# Autodesk Inventor assembly: Adrian_Box
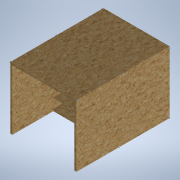
[picture p0: Inventor's stored thumbnail of the model, 180x180]
Saved by Autodesk Inventor 2021 (Build 250183000, 183)
## iProperties
Created: 2022-07-12
Part Number: Adrian_Box
Document SubType Name: Assembly
Designer: adria
Mass: 12178.9 g
Surface Area: 30264.5 cm^2
Volume: 21790.4 cm^3
Density: 0.55891 g/cm^3
Author: adria
## Documents named in this file (7)
- C:\Users\adria\OneDrive - tum.de\G2_Waste-Recycling\CAD\Adrian_Box.iam
- C:\Users\adria\OneDrive - tum.de\G2_Waste-Recycling\CAD\Seite_links.ipt
- C:\Users\adria\OneDrive - tum.de\G2_Waste-Recycling\CAD\Oben.ipt
- C:\Users\adria\OneDrive - tum.de\G2_Waste-Recycling\CAD\Seite.ipt
- C:\Users\adria\OneDrive - tum.de\G2_Waste-Recycling\CAD\Boden_drehscheibe.ipt
- C:\Users\adria\OneDrive - tum.de\G2_Waste-Recycling\CAD\Boden.ipt
- C:\Users\adria\Documents\Inventor\Content Center Files\R2021\de-DE\ANSI B18.3.1M(6)\ANSI B18.3.1M - M8x1,25 x 35(1).ipt
## Components (15 placed, 6 different names)
1. Seite_links:2 — Passend:1, Fluchtend:1, Fluchtend:2
2. Oben:1 — Passend:1, Fluchtend:1, Fluchtend:2, Fluchtend:3, Fluchtend:4, Passend:2
3. Seite:1 — Fluchtend:3, Fluchtend:4, Passend:2, Fluchtend:5, Passend:3, Fluchtend:6, Passend:4, Fluchtend:7, Passend:5, Passend:6, Passend:7, Passend:8, Passend:9, Passend:10, Passend:11, Passend:12, Passend:13, Passend:14, Fluchtend:8
4. Boden_drehscheibe:1 — Passend:4, Fluchtend:7, Passend:15
5. Boden:1 — Fluchtend:5, Passend:3, Fluchtend:6, Passend:15
6. Zylinderschraube mit geschmiedetem Innensechskant - Metrisch M8x1,25 x 35:6 — Passend:5, Passend:10
7. Zylinderschraube mit geschmiedetem Innensechskant - Metrisch M8x1,25 x 35:7 — Passend:6, Passend:11
8. Zylinderschraube mit geschmiedetem Innensechskant - Metrisch M8x1,25 x 35:8 — Passend:7, Passend:12
9. Zylinderschraube mit geschmiedetem Innensechskant - Metrisch M8x1,25 x 35:9 — Passend:9, Passend:14
10. Zylinderschraube mit geschmiedetem Innensechskant - Metrisch M8x1,25 x 35:10 — Passend:8, Passend:13
11. Zylinderschraube mit geschmiedetem Innensechskant - Metrisch M8x1,25 x 35:11
12. Zylinderschraube mit geschmiedetem Innensechskant - Metrisch M8x1,25 x 35:12
13. Zylinderschraube mit geschmiedetem Innensechskant - Metrisch M8x1,25 x 35:13
14. Zylinderschraube mit geschmiedetem Innensechskant - Metrisch M8x1,25 x 35:14
15. Zylinderschraube mit geschmiedetem Innensechskant - Metrisch M8x1,25 x 35:15
## Relationships (23: Mate 15, Flush 8)
- Passend:1 [Mate]: Seite_links:2 ↔ Oben:1
- Fluchtend:1 [Flush]: Seite_links:2 ↔ Oben:1
- Fluchtend:2 [Flush]: Seite_links:2 ↔ Oben:1
- Fluchtend:3 [Flush]: Oben:1 ↔ Seite:1
- Fluchtend:4 [Flush]: Oben:1 ↔ Seite:1
- Passend:2 [Mate]: Oben:1 ↔ Seite:1
- Fluchtend:5 [Flush]: Seite:1 ↔ Boden:1
- Passend:3 [Mate]: Seite:1 ↔ Boden:1
- Fluchtend:6 [Flush]: Seite:1 ↔ Boden:1
- Passend:4 [Mate]: Seite:1 ↔ Boden_drehscheibe:1
- Fluchtend:7 [Flush]: Seite:1 ↔ Boden_drehscheibe:1
- Passend:5 [Mate]: Seite:1 ↔ Zylinderschraube mit geschmiedetem Innensechskant - Metrisch M8x1,25 x 35:6
- Passend:6 [Mate]: Seite:1 ↔ Zylinderschraube mit geschmiedetem Innensechskant - Metrisch M8x1,25 x 35:7
- Passend:7 [Mate]: Seite:1 ↔ Zylinderschraube mit geschmiedetem Innensechskant - Metrisch M8x1,25 x 35:8
- Passend:8 [Mate]: Seite:1 ↔ Zylinderschraube mit geschmiedetem Innensechskant - Metrisch M8x1,25 x 35:10
- Passend:9 [Mate]: Seite:1 ↔ Zylinderschraube mit geschmiedetem Innensechskant - Metrisch M8x1,25 x 35:9
- Passend:10 [Mate]: Seite:1 ↔ Zylinderschraube mit geschmiedetem Innensechskant - Metrisch M8x1,25 x 35:6
- Passend:11 [Mate]: Seite:1 ↔ Zylinderschraube mit geschmiedetem Innensechskant - Metrisch M8x1,25 x 35:7
- Passend:12 [Mate]: Seite:1 ↔ Zylinderschraube mit geschmiedetem Innensechskant - Metrisch M8x1,25 x 35:8
- Passend:13 [Mate]: Seite:1 ↔ Zylinderschraube mit geschmiedetem Innensechskant - Metrisch M8x1,25 x 35:10
- Passend:14 [Mate]: Seite:1 ↔ Zylinderschraube mit geschmiedetem Innensechskant - Metrisch M8x1,25 x 35:9
- Fluchtend:8 [Flush] (-266 mm): Seite:1
- Passend:15 [Mate] (80 mm): Boden_drehscheibe:1 ↔ Boden:1
